# Autodesk Inventor assembly: IM_Matchboxscope_plate_3 MB bg
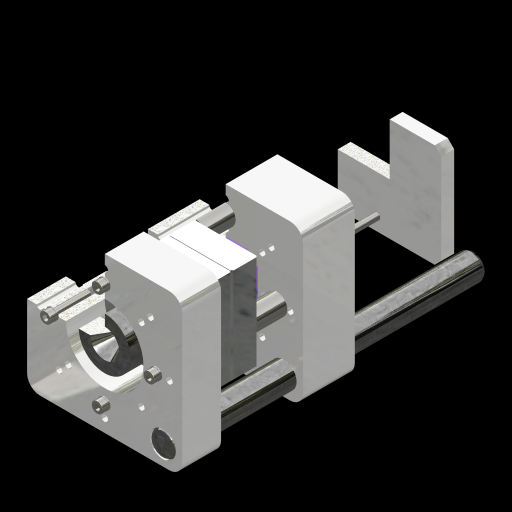
[picture p0: Inventor's stored thumbnail of the model, 512x512]
Saved by Autodesk Inventor 2024 (Build 280153000, 153)
## iProperties
Created: 2023-06-29
Part Number: IM_Matchboxscope_plate_3 MB bg
Document SubType Name: Assembly
Designer: buchmannmartin
Mass: 4335.9 g
Surface Area: 2658.93 cm^2
Volume: 1319.63 cm^3
Density: 3.28569 g/cm^3
Author: buchmannmartin
## Documents named in this file (13)
- E:\User\Dokumente\#BeneEspressoscope\IM1_Matchboxscope_plate_3 MB bg.iam
- E:\User\Dokumente\#BeneEspressoscope\MicroPlast-MB-BG.iam
- E:\User\Dokumente\#BeneEspressoscope\IM1_Matchboxscope_plate_3 MB Layout.ipt
- E:\User\Dokumente\#BeneEspressoscope\IM1_Matchboxscope_plate_3.ipt
- E:\User\Dokumente\#BeneEspressoscope\IM1-MoldTop.ipt
- E:\User\Dokumente\#BeneEspressoscope\IM1-MoldBottom.ipt
- E:\User\Dokumente\#BeneEspressoscope\Auswerfer DIN1530-AH-ISO6751-4x40mm.ipt
- E:\User\Dokumente\#BeneEspressoscope\Distanzbuchse wie MISUMI DWSSS-D16-V5-L23.ipt
- E:\User\Dokumente\Inventor\Content Center Files\R2024\de-DE\ISO 7092\ISO 7092 - ST 5 - 140 HV.ipt
- E:\User\Dokumente\Inventor\Content Center Files\R2024\de-DE\ISO 4762(2)\ISO 4762 - M5 x 45ISO.ipt
- E:\User\Dokumente\#BeneEspressoscope\Auswerfer DIN1530-AH-ISO6751-100mm.ipt
- E:\User\Dokumente\#BeneEspressoscope\D_145H_10_1\D_145H_10_1.ipt
- E:\User\Dokumente\#BeneEspressoscope\FederDummy.ipt
## Components (23 placed, 12 different names)
1. MicroPlast-MB-BG:1 [sub-assembly] — Passend:1, Passend:2, Passend:3, Passend:67, Passend:70, Passend:71, Fluchtend:8, Passend:84, Passend:85, Passend:86, Passend:87, Passend:88, Passend:89, Passend:90, Passend:91, Passend:92, Passend:94, Passend:95, Passend:96, Passend:98, Passend:99, Passend:100, Passend:101, Passend:102, Fluchtend:17
2. IM1_Matchboxscope_plate_3:1 — Fluchtend:2, Fluchtend:3, Passend:65, Passend:66, Passend:97
3. IM1-MoldTop:1 — Fluchtend:2, Fluchtend:3, Fluchtend:4, Fluchtend:5, Passend:64, Passend:66, Passend:67, Passend:68, Passend:69
4. IM1-MoldBottom:1 — Fluchtend:4, Fluchtend:5, Passend:3, Fluchtend:6, Passend:5, Passend:64, Passend:65, Fluchtend:8
5. FederDummy:2 — Passend:100, Passend:101, Passend:102, Fluchtend:17
6. IM1_Matchboxscope_plate_3 MB Layout:1 — Passend:1, Fluchtend:1, Passend:2
7. ISO 4762 M5 x 45:4 — Einfügen:4
8. ISO 4762 M5 x 45:3 — Einfügen:3
9. ISO 4762 M5 x 45:2 — Einfügen:2
10. ISO 7092 ST 5 - 140 HV:4 — Passend:91, Passend:92, Einfügen:4
11. ISO 7092 ST 5 - 140 HV:3 — Passend:89, Passend:90, Einfügen:3
12. ISO 7092 ST 5 - 140 HV:2 — Passend:87, Passend:88, Einfügen:2
13. ISO 4762 M5 x 45:1 — Einfügen:1
14. ISO 7092 ST 5 - 140 HV:1 — Passend:85, Passend:86, Einfügen:1
15. D_145H_10_1:1 — Passend:98, Passend:99
16. Auswerfer DIN1530-AH-ISO6751-100mm:2 — Fluchtend:16, Passend:93, Passend:94, Passend:96
17. Auswerfer DIN1530-AH-ISO6751-100mm:1 — Fluchtend:16, Passend:95
18. Auswerfer DIN1530-AH-ISO6751-4x40mm:1 — Passend:68, Fluchtend:7, Passend:70, Passend:71, Passend:97, Passend:93
19. Auswerfer DIN1530-AH-ISO6751-4x40mm:2 — Passend:69, Fluchtend:7
20. Distanzbuchse wie MISUMI DWSSS-D16-V5-L23:1 — Fluchtend:13, Fluchtend:14, Fluchtend:15, Passend:84
21. Distanzbuchse wie MISUMI DWSSS-D16-V5-L23:2 — Fluchtend:13
22. Distanzbuchse wie MISUMI DWSSS-D16-V5-L23:3 — Fluchtend:14
23. Distanzbuchse wie MISUMI DWSSS-D16-V5-L23:4 — Fluchtend:15
## Relationships (48: Mate 31, Flush 13, Insert 4)
- Passend:1 [Mate]: MicroPlast-MB-BG:1 ↔ IM1_Matchboxscope_plate_3 MB Layout:1
- Fluchtend:1 [Flush]: IM1_Matchboxscope_plate_3 MB Layout:1
- Passend:2 [Mate]: MicroPlast-MB-BG:1 ↔ IM1_Matchboxscope_plate_3 MB Layout:1
- Fluchtend:2 [Flush]: IM1_Matchboxscope_plate_3:1 ↔ IM1-MoldTop:1
- Fluchtend:3 [Flush]: IM1_Matchboxscope_plate_3:1 ↔ IM1-MoldTop:1
- Fluchtend:4 [Flush]: IM1-MoldTop:1 ↔ IM1-MoldBottom:1
- Fluchtend:5 [Flush]: IM1-MoldTop:1 ↔ IM1-MoldBottom:1
- Passend:3 [Mate]: MicroPlast-MB-BG:1 ↔ IM1-MoldBottom:1
- Fluchtend:6 [Flush]: IM1-MoldBottom:1
- Passend:5 [Mate]: IM1-MoldBottom:1
- Passend:64 [Mate]: IM1-MoldTop:1 ↔ IM1-MoldBottom:1
- Passend:65 [Mate]: IM1_Matchboxscope_plate_3:1 ↔ IM1-MoldBottom:1
- Passend:66 [Mate]: IM1_Matchboxscope_plate_3:1 ↔ IM1-MoldTop:1
- Passend:67 [Mate]: MicroPlast-MB-BG:1 ↔ IM1-MoldTop:1
- Passend:68 [Mate]: IM1-MoldTop:1 ↔ Auswerfer DIN1530-AH-ISO6751-4x40mm:1
- Passend:69 [Mate]: IM1-MoldTop:1 ↔ Auswerfer DIN1530-AH-ISO6751-4x40mm:2
- Fluchtend:7 [Flush]: Auswerfer DIN1530-AH-ISO6751-4x40mm:1 ↔ Auswerfer DIN1530-AH-ISO6751-4x40mm:2
- Passend:70 [Mate]: MicroPlast-MB-BG:1 ↔ Auswerfer DIN1530-AH-ISO6751-4x40mm:1
- Passend:71 [Mate]: MicroPlast-MB-BG:1 ↔ Auswerfer DIN1530-AH-ISO6751-4x40mm:1
- Fluchtend:8 [Flush] (180 mm): MicroPlast-MB-BG:1 ↔ IM1-MoldBottom:1
- Fluchtend:13 [Flush]: Distanzbuchse wie MISUMI DWSSS-D16-V5-L23:1 ↔ Distanzbuchse wie MISUMI DWSSS-D16-V5-L23:2
- Fluchtend:14 [Flush]: Distanzbuchse wie MISUMI DWSSS-D16-V5-L23:1 ↔ Distanzbuchse wie MISUMI DWSSS-D16-V5-L23:3
- Fluchtend:15 [Flush]: Distanzbuchse wie MISUMI DWSSS-D16-V5-L23:1 ↔ Distanzbuchse wie MISUMI DWSSS-D16-V5-L23:4
- Passend:84 [Mate]: MicroPlast-MB-BG:1 ↔ Distanzbuchse wie MISUMI DWSSS-D16-V5-L23:1
- Passend:85 [Mate]: MicroPlast-MB-BG:1 ↔ ISO 7092 ST 5 - 140 HV:1
- Passend:86 [Mate]: MicroPlast-MB-BG:1 ↔ ISO 7092 ST 5 - 140 HV:1
- Passend:87 [Mate]: MicroPlast-MB-BG:1 ↔ ISO 7092 ST 5 - 140 HV:2
- Passend:88 [Mate]: MicroPlast-MB-BG:1 ↔ ISO 7092 ST 5 - 140 HV:2
- Passend:89 [Mate]: MicroPlast-MB-BG:1 ↔ ISO 7092 ST 5 - 140 HV:3
- Passend:90 [Mate]: MicroPlast-MB-BG:1 ↔ ISO 7092 ST 5 - 140 HV:3
- Passend:91 [Mate]: MicroPlast-MB-BG:1 ↔ ISO 7092 ST 5 - 140 HV:4
- Passend:92 [Mate]: MicroPlast-MB-BG:1 ↔ ISO 7092 ST 5 - 140 HV:4
- Einfügen:1 [Insert]: ISO 4762 M5 x 45:1 ↔ ISO 7092 ST 5 - 140 HV:1
- Einfügen:2 [Insert]: ISO 4762 M5 x 45:2 ↔ ISO 7092 ST 5 - 140 HV:2
- Einfügen:3 [Insert]: ISO 4762 M5 x 45:3 ↔ ISO 7092 ST 5 - 140 HV:3
- Einfügen:4 [Insert]: ISO 4762 M5 x 45:4 ↔ ISO 7092 ST 5 - 140 HV:4
- Fluchtend:16 [Flush]: Auswerfer DIN1530-AH-ISO6751-100mm:2 ↔ Auswerfer DIN1530-AH-ISO6751-100mm:1
- Passend:93 [Mate]: Auswerfer DIN1530-AH-ISO6751-100mm:2 ↔ Auswerfer DIN1530-AH-ISO6751-4x40mm:1
- Passend:94 [Mate]: MicroPlast-MB-BG:1 ↔ Auswerfer DIN1530-AH-ISO6751-100mm:2
- Passend:95 [Mate]: MicroPlast-MB-BG:1 ↔ Auswerfer DIN1530-AH-ISO6751-100mm:1
- Passend:96 [Mate]: MicroPlast-MB-BG:1 ↔ Auswerfer DIN1530-AH-ISO6751-100mm:2
- Passend:97 [Mate] (0.2 mm): IM1_Matchboxscope_plate_3:1 ↔ Auswerfer DIN1530-AH-ISO6751-4x40mm:1
- Passend:98 [Mate]: MicroPlast-MB-BG:1 ↔ D_145H_10_1:1
- Passend:99 [Mate]: MicroPlast-MB-BG:1 ↔ D_145H_10_1:1
- Passend:100 [Mate]: MicroPlast-MB-BG:1 ↔ FederDummy:2
- Passend:101 [Mate]: MicroPlast-MB-BG:1 ↔ FederDummy:2
- Passend:102 [Mate]: MicroPlast-MB-BG:1 ↔ FederDummy:2
- Fluchtend:17 [Flush] (17 mm): MicroPlast-MB-BG:1 ↔ FederDummy:2
